# Autodesk Inventor assembly: A2017_T3_01
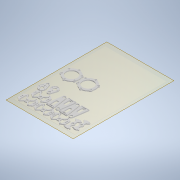
[picture p0: Inventor's stored thumbnail of the model, 180x180]
Saved by Autodesk Inventor 2020 (Build 240168000, 168)
## iProperties
Created: 2021-08-27
Part Number: A2017_T3_01
Document SubType Name: Assembly
Designer: Masato
Author: Masato
## Documents named in this file (7)
- C:\Users\marin\Documents\0118 git clone\OpenPlatform_ver3_0\cam\A2017_T3_01.iam
- C:\Users\marin\Documents\0118 git clone\OpenPlatform_ver3_0\cam\Disposable_Board.ipt
- C:\Users\marin\Documents\0118 git clone\OpenPlatform_ver3_0\LowerBody\Leg_joit\Leg_joint_slider_frame.ipt
- C:\Users\marin\Documents\0118 git clone\OpenPlatform_ver3_0\LowerBody\Leg_joit\Leg_joint_roll_frame.ipt
- C:\Users\marin\Documents\0118 git clone\OpenPlatform_ver3_0\LowerBody\Slider_crank\Slider_crank_horn.ipt
- C:\Users\marin\Documents\0118 git clone\OpenPlatform_ver3_0\LowerBody\Ankle\Ankle_front_frame.ipt
- C:\Users\marin\Documents\0118 git clone\OpenPlatform_ver3_0\UpperBody\Trunk\CrossRollerBearing\Outer_flange.ipt
## Components (15 placed, 6 different names)
1. Disposable_Board:1 — メイト:2, メイト:1, フラッシュ:1, フラッシュ:2, フラッシュ:3, 正接:1, 正接:2, 正接:3, フラッシュ:5, フラッシュ:7, 正接:9, 角度:1, 角度:2, 正接:13, 正接:14
2. Leg_joint_slider_frame:1 — メイト:4, メイト:18, 正接:5, 正接:6, メイト:19
3. Leg_joint_slider_frame:2 — メイト:5, メイト:21, 正接:8
4. Leg_joint_slider_frame:3 — メイト:7, メイト:20, 正接:7, メイト:21, 正接:8
5. Leg_joint_slider_frame:4 — メイト:6, 正接:6, メイト:19, メイト:20, 正接:7
6. Leg_joint_roll_frame:1 — メイト:8, フラッシュ:3, 正接:1, メイト:16, フラッシュ:4, 正接:12
7. Leg_joint_roll_frame:2 — メイト:10, メイト:16, 正接:2, メイト:17, 正接:5
8. Leg_joint_roll_frame:3 — メイト:11, メイト:17, 正接:3, メイト:22
9. Leg_joint_roll_frame:4 — メイト:9, フラッシュ:4, メイト:18, 正接:10, 正接:11, 正接:12
10. Slider_crank_horn:1 — メイト:14, 正接:9, 正接:10, メイト:23, 角度:1
11. Slider_crank_horn:2 — メイト:15, メイト:23, 正接:11
12. Ankle_front_frame:1 — メイト:13, フラッシュ:5, メイト:22, フラッシュ:6
13. Ankle_front_frame:2 — メイト:12, フラッシュ:6, フラッシュ:7
14. Outer_flange:1 — メイト:24, 角度:2, 正接:13, 正接:14
15. Outer_flange:2
## Component patterns: (2 elements, first: Outer_flange:1)
## Relationships (45: Mate 23, Tangent 13, Flush 7, Angle 2)
- メイト:2 [Mate]: Disposable_Board:1
- メイト:1 [Mate]: Disposable_Board:1
- フラッシュ:1 [Flush]: Disposable_Board:1
- フラッシュ:2 [Flush]: Disposable_Board:1
- メイト:4 [Mate]: Leg_joint_slider_frame:1
- メイト:5 [Mate]: Leg_joint_slider_frame:2
- メイト:6 [Mate]: Leg_joint_slider_frame:4
- メイト:7 [Mate]: Leg_joint_slider_frame:3
- メイト:8 [Mate]: Leg_joint_roll_frame:1
- メイト:9 [Mate]: Leg_joint_roll_frame:4
- メイト:10 [Mate]: Leg_joint_roll_frame:2
- メイト:11 [Mate]: Leg_joint_roll_frame:3
- メイト:12 [Mate]: Ankle_front_frame:2
- メイト:13 [Mate]: Ankle_front_frame:1
- メイト:14 [Mate]: Slider_crank_horn:1
- メイト:15 [Mate]: Slider_crank_horn:2
- フラッシュ:3 [Flush] (3 mm): Disposable_Board:1 ↔ Leg_joint_roll_frame:1
- 正接:1 [Tangent] (3 mm): Disposable_Board:1 ↔ Leg_joint_roll_frame:1
- メイト:16 [Mate] (3 mm): Leg_joint_roll_frame:1 ↔ Leg_joint_roll_frame:2
- 正接:2 [Tangent] (3 mm): Disposable_Board:1 ↔ Leg_joint_roll_frame:2
- メイト:17 [Mate] (3 mm): Leg_joint_roll_frame:2 ↔ Leg_joint_roll_frame:3
- 正接:3 [Tangent] (3 mm): Disposable_Board:1 ↔ Leg_joint_roll_frame:3
- フラッシュ:4 [Flush] (12 mm): Leg_joint_roll_frame:1 ↔ Leg_joint_roll_frame:4
- メイト:18 [Mate] (3 mm): Leg_joint_slider_frame:1 ↔ Leg_joint_roll_frame:4
- 正接:5 [Tangent] (3 mm): Leg_joint_slider_frame:1 ↔ Leg_joint_roll_frame:2
- 正接:6 [Tangent]: Leg_joint_slider_frame:1 ↔ Leg_joint_slider_frame:4
- メイト:19 [Mate] (3 mm): Leg_joint_slider_frame:1 ↔ Leg_joint_slider_frame:4
- メイト:20 [Mate] (3 mm): Leg_joint_slider_frame:3 ↔ Leg_joint_slider_frame:4
- 正接:7 [Tangent]: Leg_joint_slider_frame:3 ↔ Leg_joint_slider_frame:4
- メイト:21 [Mate] (3 mm): Leg_joint_slider_frame:2 ↔ Leg_joint_slider_frame:3
- 正接:8 [Tangent]: Leg_joint_slider_frame:2 ↔ Leg_joint_slider_frame:3
- フラッシュ:5 [Flush] (3 mm): Disposable_Board:1 ↔ Ankle_front_frame:1
- メイト:22 [Mate] (8 mm): Leg_joint_roll_frame:3 ↔ Ankle_front_frame:1
- フラッシュ:6 [Flush] (-10 mm): Ankle_front_frame:1 ↔ Ankle_front_frame:2
- フラッシュ:7 [Flush] (3 mm): Disposable_Board:1 ↔ Ankle_front_frame:2
- 正接:9 [Tangent] (4 mm): Disposable_Board:1 ↔ Slider_crank_horn:1
- 正接:10 [Tangent] (3 mm): Leg_joint_roll_frame:4 ↔ Slider_crank_horn:1
- メイト:23 [Mate] (6 mm): Slider_crank_horn:1 ↔ Slider_crank_horn:2
- 正接:11 [Tangent] (3 mm): Leg_joint_roll_frame:4 ↔ Slider_crank_horn:2
- 正接:12 [Tangent]: Leg_joint_roll_frame:1 ↔ Leg_joint_roll_frame:4
- 角度:1 [Angle] (0 deg): Disposable_Board:1 ↔ Slider_crank_horn:1
- メイト:24 [Mate]: Outer_flange:1
- 角度:2 [Angle] (0 deg): Disposable_Board:1 ↔ Outer_flange:1
- 正接:13 [Tangent] (3 mm): Disposable_Board:1 ↔ Outer_flange:1
- 正接:14 [Tangent] (110 mm): Disposable_Board:1 ↔ Outer_flange:1
